# Autodesk Inventor assembly: Assembly10
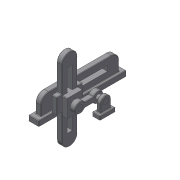
[picture p0: Inventor's stored thumbnail of the model, 180x180]
Saved by Autodesk Inventor 2017 (Build 210142000, 142)
## iProperties
Created: 2016-07-28
Part Number: Assembly10
Document SubType Name: Assembly
Designer: Tutorial Books
Author: Tutorial Books
## Documents named in this file (7)
- C:\Users\anand\Documents\Inventor\Autodesk Inventor 2017 Learn by doing\Slider Crank Mechanism\Assembly10.iam
- C:\Users\anand\Documents\Inventor\Autodesk Inventor 2017 Learn by doing\Slider Crank Mechanism\Base.ipt
- C:\Users\anand\Documents\Inventor\Autodesk Inventor 2017 Learn by doing\Slider Crank Mechanism\Arm.ipt
- C:\Users\anand\Documents\Inventor\Autodesk Inventor 2017 Learn by doing\Slider Crank Mechanism\Pin.ipt
- C:\Users\anand\Documents\Inventor\Autodesk Inventor 2017 Learn by doing\Slider Crank Mechanism\Pivot.ipt
- C:\Users\anand\Documents\Inventor\Autodesk Inventor 2017 Learn by doing\Slider Crank Mechanism\Slider1.ipt
- C:\Users\anand\Documents\Inventor\Autodesk Inventor 2017 Learn by doing\Slider Crank Mechanism\Slider2.ipt
## Components (6 placed, 6 different names)
1. Base:1 — Slider:1, Flush:1, Flush:2
2. Arm:1 — Rotational:1, Rigid:1
3. Pin:1 — Rigid:1, Rotational:2
4. Pivot:1 — Rotational:2, Flush:1, Flush:2
5. Slider1:1 — Slider:1, Slider:2
6. Slider2:1 — Slider:2, Rotational:1
## Relationships (7: TranslationJoint 2, RevoluteJoint 2, Flush 2, WeldJoint 1)
- Slider:1 [TranslationJoint]: Base:1 ↔ Slider1:1
- Slider:2 [TranslationJoint]: Slider1:1 ↔ Slider2:1
- Rotational:1 [RevoluteJoint]: Arm:1 ↔ Slider2:1
- Rigid:1 [WeldJoint]: Arm:1 ↔ Pin:1
- Rotational:2 [RevoluteJoint]: Pin:1 ↔ Pivot:1
- Flush:1: Base:1 ↔ Pivot:1
- Flush:2: Base:1 ↔ Pivot:1
